# Autodesk Inventor assembly: Bumpers
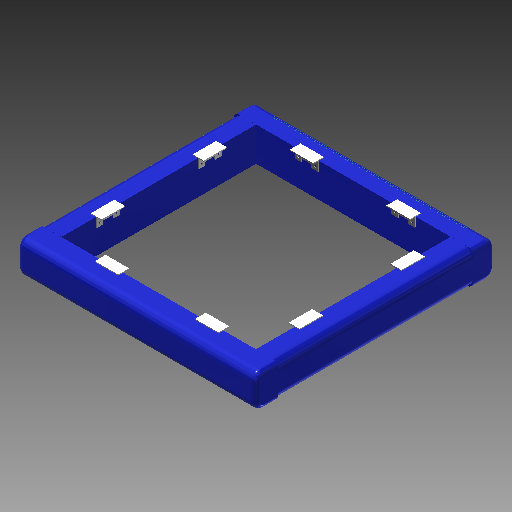
[picture p0: Inventor's stored thumbnail of the model, 512x512]
Saved by Autodesk Inventor 2018.3 (Build 223284000, 284)
## iProperties
Created: 2020-02-05
Part Number: Bumpers
Document SubType Name: Assembly
Designer: Myers
Author: Myers
## Documents named in this file (4)
- C:\Users\22turnmaxw\Documents\GrabCAD\Infinite Recharge 2020\Build season\Bumper\Bumpers.iam
- C:\Users\22turnmaxw\Documents\GrabCAD\Infinite Recharge 2020\Build season\Bumper\FBBumper.ipt
- C:\Users\22turnmaxw\Documents\GrabCAD\Infinite Recharge 2020\Build season\Bumper\SideBumper.ipt
- C:\Users\22turnmaxw\Documents\GrabCAD\Infinite Recharge 2020\Build season\Bumper\t 2 piece.ipt
## Components (12 placed, 3 different names)
1. SideBumper:1 — Mate:1, Flush:1, Flush:2, Flush:3, Mate:2, Flush:4, Flush:5, Mate:4, Mate:5, Mate:6
2. FBBumper:1 — Mate:1, Flush:1, Mate:3, Flush:4, Mate:9, Mate:10
3. FBBumper:2 — Flush:3, Mate:2, Flush:5, Flush:6, Mate:7, Mate:8
4. SideBumper:2 — Flush:2, Mate:3, Flush:6, Mate:11, Mate:12
5. t 2 piece:1 — Flush:7, Mate:6
6. t 2 piece:2 — Mate:4, Mate:5, Flush:7, Flush:8, Flush:9, Flush:10, Flush:11, Flush:12, Flush:13
7. t 2 piece:3 — Mate:7, Flush:9
8. t 2 piece:4 — Mate:8, Flush:8
9. t 2 piece:5 — Flush:10, Mate:12
10. t 2 piece:6 — Flush:11, Mate:11
11. t 2 piece:7 — Flush:12, Mate:9
12. t 2 piece:8 — Flush:13, Mate:10
## Relationships (25: Flush 13, Mate 12)
- Mate:1: SideBumper:1 ↔ FBBumper:1
- Flush:1: SideBumper:1 ↔ FBBumper:1
- Flush:2: SideBumper:1 ↔ SideBumper:2
- Flush:3: SideBumper:1 ↔ FBBumper:2
- Mate:2: SideBumper:1 ↔ FBBumper:2
- Mate:3: FBBumper:1 ↔ SideBumper:2
- Flush:4: SideBumper:1 ↔ FBBumper:1
- Flush:5: SideBumper:1 ↔ FBBumper:2
- Flush:6: FBBumper:2 ↔ SideBumper:2
- Mate:4: SideBumper:1 ↔ t 2 piece:2
- Mate:5: SideBumper:1 ↔ t 2 piece:2
- Flush:7: t 2 piece:1 ↔ t 2 piece:2
- Mate:6: SideBumper:1 ↔ t 2 piece:1
- Mate:7: FBBumper:2 ↔ t 2 piece:3
- Mate:8: FBBumper:2 ↔ t 2 piece:4
- Flush:8: t 2 piece:2 ↔ t 2 piece:4
- Flush:9: t 2 piece:2 ↔ t 2 piece:3
- Flush:10: t 2 piece:2 ↔ t 2 piece:5
- Flush:11: t 2 piece:2 ↔ t 2 piece:6
- Flush:12: t 2 piece:2 ↔ t 2 piece:7
- Flush:13: t 2 piece:2 ↔ t 2 piece:8
- Mate:9: FBBumper:1 ↔ t 2 piece:7
- Mate:10: FBBumper:1 ↔ t 2 piece:8
- Mate:11: SideBumper:2 ↔ t 2 piece:6
- Mate:12: SideBumper:2 ↔ t 2 piece:5
